# Autodesk Inventor assembly: wheel
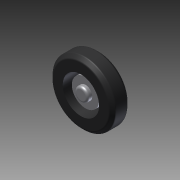
[picture p0: Inventor's stored thumbnail of the model, 180x180]
Saved by Autodesk Inventor 2012 (Build 160160000, 160)
## iProperties
Created: 2011-10-06
Part Number: wheel
Document SubType Name: Assembly
Designer: Antonella
Author: Antonella
## Documents named in this file (3)
- C:\Users\Antonella\Documents\GCC Robotics 2012 - Mechanical\Version 2\Drive Train\Wheel\wheel.iam
- C:\Users\Antonella\Documents\GCC Robotics 2012 - Mechanical\Version 2\Drive Train\Wheel\wheel.ipt
- C:\Users\Antonella\Documents\GCC Robotics 2012 - Mechanical\Version 2\Drive Train\Wheel\tire.ipt
## Components (2 placed, 2 different names)
1. wheel:1 — Mate:1, Flush:1
2. tire:1 — Mate:1, Flush:1
## Relationships (2: Mate 1, Flush 1)
- Mate:1: wheel:1 ↔ tire:1
- Flush:1: wheel:1 ↔ tire:1
